# Autodesk Inventor assembly: RevSingleStage
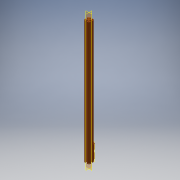
[picture p0: Inventor's stored thumbnail of the model, 180x180]
Saved by Autodesk Inventor 2018 (Build 220112000, 112)
## iProperties
Created: 2017-11-25
Part Number: RevSingleStage
Document SubType Name: Assembly
Designer: ball
Author: ball
## Documents named in this file (3)
- C:\FTC\FTC8863CAD\2017Robot\RevSingleStage.iam
- C:\FTC\FTC8863CAD\RevRobotics\REV-41-1017_15mm_extrusion_17.875in.ipt
- C:\FTC\FTC8863CAD\RevRobotics\REV-41-1094.ipt
## Components (2 placed, 2 different names)
1. REV-41-1017_15mm_extrusion_17.875in:2 — Mate:5, Mate:6, Flush:5
2. REV-41-1094:1 — Mate:5, Mate:6, Flush:5
## Relationships (3: Mate 2, Flush 1)
- Mate:5: REV-41-1017_15mm_extrusion_17.875in:2 ↔ REV-41-1094:1
- Mate:6: REV-41-1017_15mm_extrusion_17.875in:2 ↔ REV-41-1094:1
- Flush:5: REV-41-1017_15mm_extrusion_17.875in:2 ↔ REV-41-1094:1
